# Autodesk Inventor assembly: section_rod
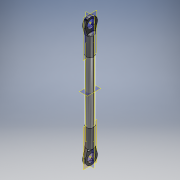
[picture p0: Inventor's stored thumbnail of the model, 180x180]
Saved by Autodesk Inventor 2017 (Build 210142000, 142)
## iProperties
Part Number: section_rod
Material: Ogólny
Document SubType Name: Assembly
Designer: Speed King
Mass: 2.29242 g
Surface Area: 20.9483 cm^2
Volume: 2.22383 cm^3
Density: 1.03084 g/cm^3
Author: Speed King
## Documents named in this file (3)
- C:\Users\Speed King\Documents\My Inventor\GrabCAD\Technical Informatics\CAD\model\section_rod.iam
- C:\Users\Speed King\Documents\My Inventor\GrabCAD\Technical Informatics\CAD\model\rod.ipt
- C:\Users\Speed King\Documents\My Inventor\GrabCAD\Technical Informatics\CAD\model\joint_body.ipt
## Components (3 placed, 2 different names)
1. rod:1 — Zestawiający:1, Zestawiający:2, Zestawiający:3, Zestawiający:4, Zestawiający:5, Zestawiający:6, Zestawiający:8, Zestawiający:9
2. joint_body:1 — Zestawiający:1, Zestawiający:2, Zestawiający:5, Symetria:1
3. joint_body:2 — Zestawiający:3, Zestawiający:4, Zestawiający:6, Symetria:1
## Relationships (10: Mate 9, Symmetry 1)
- Zestawiający:1 [Mate]: rod:1 ↔ joint_body:1
- Zestawiający:2 [Mate]: rod:1 ↔ joint_body:1
- Zestawiający:3 [Mate]: rod:1 ↔ joint_body:2
- Zestawiający:4 [Mate]: rod:1 ↔ joint_body:2
- Zestawiający:5 [Mate]: rod:1 ↔ joint_body:1
- Zestawiający:6 [Mate]: rod:1 ↔ joint_body:2
- Zestawiający:8 [Mate]: rod:1
- Zestawiający:9 [Mate]: rod:1
- Symetria:1 [Symmetry]: joint_body:1 ↔ joint_body:2
- Zestawiający:10 [Mate]
